# Autodesk Inventor assembly: FRONT FRAME ASSEMBLY
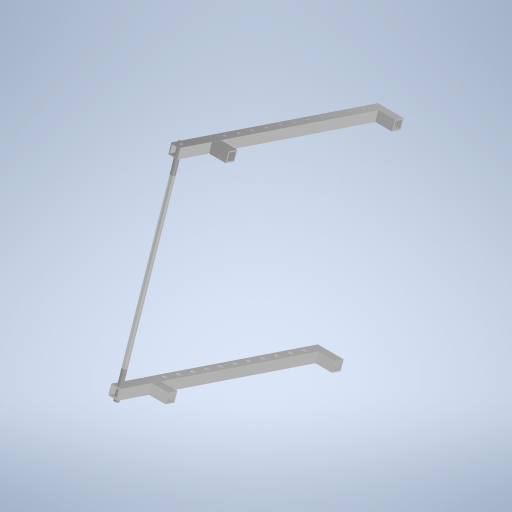
[picture p0: Inventor's stored thumbnail of the model, 512x512]
Saved by Autodesk Inventor 2023 (Build 270158000, 158)
## iProperties
Created: 2022-08-29
Part Number: FRONT FRAME ASSEMBLY
Document SubType Name: Assembly
Designer: D.C. Eksteen
Author: D.C. Eksteen
## Documents named in this file (4)
- C:\Users\dylan\Desktop\Skripsie-2022\Design\CAD\FRONT FRAME ASSEMBLY.iam
- C:\Users\dylan\Desktop\Skripsie-2022\Design\CAD\FRONT FRAME LEFT.iam
- C:\Users\dylan\Desktop\Skripsie-2022\Design\CAD\FRONT FRAME HINGE ROD.ipt
- C:\Users\dylan\Desktop\Skripsie-2022\Design\CAD\FRONT FRAME RIGHT.iam
## Components (3 placed, 3 different names)
1. FRONT FRAME LEFT:1 [sub-assembly]
2. FRONT FRAME HINGE ROD:1
3. FRONT FRAME RIGHT:1 [sub-assembly]
## Relationships (4: Mate 3, Flush 1)
- [Mate]: FRONT FRAME LEFT:1 ↔ FRONT FRAME HINGE ROD:1
- [Mate]: FRONT FRAME HINGE ROD:1 ↔ FRONT FRAME RIGHT:1
- [Flush]: FRONT FRAME LEFT:1 ↔ FRONT FRAME RIGHT:1
- [Mate] (530 mm): FRONT FRAME LEFT:1 ↔ FRONT FRAME RIGHT:1
